# Autodesk Inventor assembly: KB33-046-002 - Рама
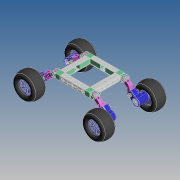
[picture p0: Inventor's stored thumbnail of the model, 180x180]
Saved by Autodesk Inventor 2020 (Build 240168000, 168)
## iProperties
Created: 2021-06-09
Part Number: KB33-046-002 - Рама
Material: Типовые
Document SubType Name: Assembly
Designer: Петров Иван
Mass: 6033.98 g
Surface Area: 9331.19 cm^2
Volume: 5518.72 cm^3
Density: 1.09337 g/cm^3
Author: Петров Иван
## Documents named in this file (4)
- E:\IVAN\Ivan_desktop\Kvantorium\Projects\RoboPatrol\design\KB33-046-001 - Ходовая часть.iam
- E:\IVAN\Ivan_desktop\Kvantorium\Projects\RoboPatrol\design\standart_components\Tetrix\ftc-tetrix-kit-of-parts-1.snapshot.34\MAX Channels\160mm Channel.ipt
- E:\IVAN\Ivan_desktop\Kvantorium\Projects\RoboPatrol\design\KB33-046-002 - Уголок с креплением мотора.iam
- E:\IVAN\Ivan_desktop\Kvantorium\Projects\RoboPatrol\design\KB33-046-002 - Уголок с креплением мотора1.iam
## Components (8 placed, 3 different names)
1. 160mm Channel:2 — Совмещение:1, Совмещение:5, Совмещение:11
2. 160mm Channel:3 — Совмещение:2, Совмещение:3, Совмещение:10, Заподлицо:2
3. 160mm Channel:4 — Совмещение:6, Совмещение:7, Совмещение:9
4. 160mm Channel:5 — Совмещение:4, Совмещение:8, Заподлицо:1
5. KB33-046-002 - Уголок с креплением мотора:1 [sub-assembly] — Совмещение:2, Совмещение:3, Совмещение:4
6. KB33-046-002 - Уголок с креплением мотора:2 [sub-assembly] — Совмещение:5, Совмещение:6, Совмещение:7
7. KB33-046-002 - Уголок с креплением мотора1:1 [sub-assembly] — Совмещение:8, Совмещение:9, Заподлицо:1
8. KB33-046-002 - Уголок с креплением мотора1:2 [sub-assembly] — Совмещение:10, Совмещение:11, Заподлицо:2
## Relationships (13: Mate 11, Flush 2)
- Совмещение:1 [Mate]: 160mm Channel:2
- Совмещение:2 [Mate]: 160mm Channel:3 ↔ KB33-046-002 - Уголок с креплением мотора:1
- Совмещение:3 [Mate]: 160mm Channel:3 ↔ KB33-046-002 - Уголок с креплением мотора:1
- Совмещение:4 [Mate]: 160mm Channel:5 ↔ KB33-046-002 - Уголок с креплением мотора:1
- Совмещение:5 [Mate]: 160mm Channel:2 ↔ KB33-046-002 - Уголок с креплением мотора:2
- Совмещение:6 [Mate]: 160mm Channel:4 ↔ KB33-046-002 - Уголок с креплением мотора:2
- Совмещение:7 [Mate]: 160mm Channel:4 ↔ KB33-046-002 - Уголок с креплением мотора:2
- Совмещение:8 [Mate]: 160mm Channel:5 ↔ KB33-046-002 - Уголок с креплением мотора1:1
- Совмещение:9 [Mate]: 160mm Channel:4 ↔ KB33-046-002 - Уголок с креплением мотора1:1
- Заподлицо:1 [Flush]: 160mm Channel:5 ↔ KB33-046-002 - Уголок с креплением мотора1:1
- Совмещение:10 [Mate]: 160mm Channel:3 ↔ KB33-046-002 - Уголок с креплением мотора1:2
- Совмещение:11 [Mate]: 160mm Channel:2 ↔ KB33-046-002 - Уголок с креплением мотора1:2
- Заподлицо:2 [Flush]: 160mm Channel:3 ↔ KB33-046-002 - Уголок с креплением мотора1:2
